# Autodesk Inventor assembly: hc-sr04
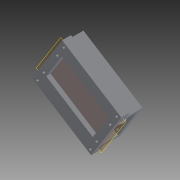
[picture p0: Inventor's stored thumbnail of the model, 180x180]
Saved by Autodesk Inventor 2015 (Build 190159000, 159)
## iProperties
Created: 2015-03-05
Part Number: hc-sr04
Document SubType Name: Assembly
Designer: ChristopherEvan
Author: Christoper Allemang
Title: C:\Users\Christoper Allemang\Documents\MAKE\Arduino Kit CAD Library\Step\HC-SR04.stp
Creation Date: 2014-09-10
Sending System: Autodesk Inventor 2015
Preprocessor: ST-DEVELOPER v15.6
Author: ChristopherEvan
## Documents named in this file (4)
- C:\Users\ChristopherEvan\Documents\Inventor\MAKE\Enclosure\ProxSensor\hc-sr04.iam
- C:\Users\ChristopherEvan\Documents\Inventor\MAKE\Enclosure\ProxSensor\UltraSonic.ipt
- C:\Users\ChristopherEvan\Documents\Inventor\MAKE\Enclosure\ProxSensor\ProxSensor_Bracket.ipt
- C:\Users\ChristopherEvan\Documents\Inventor\MAKE\Enclosure\ProxSensor\ProxSensor_Bracket_Back.ipt
## Components (3 placed, 3 different names)
1. UltraSonic_2 — Mate:1, Mate:2, Mate:3, Mate:4, Mate:5
2. ProxSensor_Bracket_Back:1 — Mate:1, Mate:2, Mate:3, Mate:6
3. ProxSensor_Bracket:1 — Mate:4, Mate:5, Mate:6
## Relationships (6: Mate 6)
- Mate:1: UltraSonic_2 ↔ ProxSensor_Bracket_Back:1
- Mate:2: UltraSonic_2 ↔ ProxSensor_Bracket_Back:1
- Mate:3: UltraSonic_2 ↔ ProxSensor_Bracket_Back:1
- Mate:4: UltraSonic_2 ↔ ProxSensor_Bracket:1
- Mate:5: UltraSonic_2 ↔ ProxSensor_Bracket:1
- Mate:6: ProxSensor_Bracket_Back:1 ↔ ProxSensor_Bracket:1
